# Autodesk Inventor assembly: jukebis SQ M
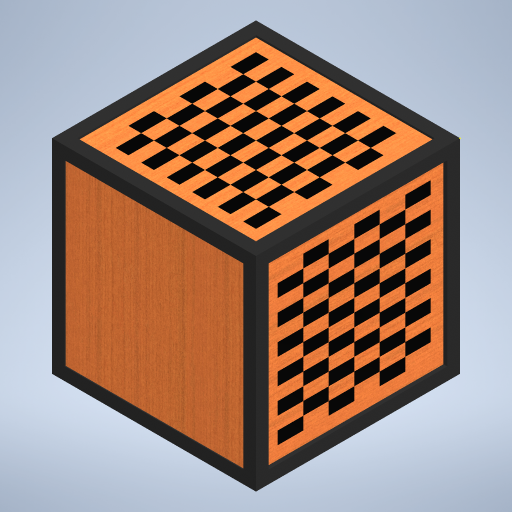
[picture p0: Inventor's stored thumbnail of the model, 512x512]
Saved by Autodesk Inventor 2024 (Build 280153000, 153)
## iProperties
Created: 2023-05-30
Part Number: jukebis SQ M
Document SubType Name: Assembly
Designer: newic
Author: newic
## Documents named in this file (7)
- D:\.My Models\.Inventor\Jukebox Project\jukebis SQ M.iam
- D:\.My Models\.Inventor\Jukebox Project\JukeBox Bottem Panel.ipt
- D:\.My Models\.Inventor\Jukebox Project\JukeBox CD Player SQ.ipt
- D:\.My Models\.Inventor\Jukebox Project\JukeBox Metal Frame.ipt
- D:\.My Models\.Inventor\Jukebox Project\JukeBox Outside panel sharp edges magnet slit.ipt
- D:\.My Models\.Inventor\Jukebox Project\JukeBox Top Panel SQ.ipt
- D:\.My Models\.Inventor\Jukebox Project\Mesh.ipt
## Components (12 placed, 6 different names)
1. JukeBox Bottem Panel:1 — Mate:7, Mate:8, Mate:16, Mate:20, Mate:21, Mate:22
2. JukeBox CD Player SQ:1 — Mate:12, Mate:13
3. JukeBox Metal Frame:1 — Mate:1, Mate:2, Mate:3, Mate:4, Mate:5, Mate:6, Mate:7, Mate:8, Mate:9, Mate:10, Mate:11, Mate:14
4. JukeBox Outside panel sharp edges magnet slit:1 — Mate:6, Mate:10, Mate:19
5. JukeBox Outside panel sharp edges magnet slit:2 — Mate:4, Mate:9, Mate:18
6. JukeBox Outside panel sharp edges magnet slit:3 — Mate:3, Mate:14, Mate:17
7. JukeBox Outside panel sharp edges magnet slit:4 — Mate:5, Mate:11, Mate:15
8. JukeBox Top Panel SQ:1 — Mate:1, Mate:2, Mate:12, Mate:13
9. Mesh:1 — Mate:19, Mate:21
10. Mesh:2 — Mate:18, Mate:22
11. Mesh:3 — Mate:17, Mate:20
12. Mesh:4 — Mate:15, Mate:16
## Relationships (22: Mate 22)
- Mate:1: JukeBox Metal Frame:1 ↔ JukeBox Top Panel SQ:1
- Mate:2: JukeBox Metal Frame:1 ↔ JukeBox Top Panel SQ:1
- Mate:3: JukeBox Metal Frame:1 ↔ JukeBox Outside panel sharp edges magnet slit:3
- Mate:4: JukeBox Metal Frame:1 ↔ JukeBox Outside panel sharp edges magnet slit:2
- Mate:5: JukeBox Metal Frame:1 ↔ JukeBox Outside panel sharp edges magnet slit:4
- Mate:6: JukeBox Metal Frame:1 ↔ JukeBox Outside panel sharp edges magnet slit:1
- Mate:7: JukeBox Bottem Panel:1 ↔ JukeBox Metal Frame:1
- Mate:8: JukeBox Bottem Panel:1 ↔ JukeBox Metal Frame:1
- Mate:9: JukeBox Metal Frame:1 ↔ JukeBox Outside panel sharp edges magnet slit:2
- Mate:10: JukeBox Metal Frame:1 ↔ JukeBox Outside panel sharp edges magnet slit:1
- Mate:11: JukeBox Metal Frame:1 ↔ JukeBox Outside panel sharp edges magnet slit:4
- Mate:12: JukeBox CD Player SQ:1 ↔ JukeBox Top Panel SQ:1
- Mate:13: JukeBox CD Player SQ:1 ↔ JukeBox Top Panel SQ:1
- Mate:14: JukeBox Metal Frame:1 ↔ JukeBox Outside panel sharp edges magnet slit:3
- Mate:15: JukeBox Outside panel sharp edges magnet slit:4 ↔ Mesh:4
- Mate:16: JukeBox Bottem Panel:1 ↔ Mesh:4
- Mate:17: JukeBox Outside panel sharp edges magnet slit:3 ↔ Mesh:3
- Mate:18: JukeBox Outside panel sharp edges magnet slit:2 ↔ Mesh:2
- Mate:19: JukeBox Outside panel sharp edges magnet slit:1 ↔ Mesh:1
- Mate:20: JukeBox Bottem Panel:1 ↔ Mesh:3
- Mate:21: JukeBox Bottem Panel:1 ↔ Mesh:1
- Mate:22: JukeBox Bottem Panel:1 ↔ Mesh:2
